# Autodesk Inventor assembly: 00_033_BATTERY_LIB_R1
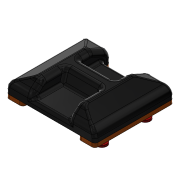
[picture p0: Inventor's stored thumbnail of the model, 180x180]
Saved by Autodesk Inventor 2021.2 (Build 252289000, 289)
## iProperties
Created: 2018-09-07
Part Number: 00_033_BATTERY_LIB_R1
Material: 一般
Document SubType Name: Assembly
Designer: y6tada
Author: y6tada
## Documents named in this file (4)
- C:\Workspace\HaptHexa\Hardware\Inventor\00_033_BATTERY_LIB_R1.iam
- C:\Workspace\HaptHexa\Hardware\Inventor\15_037_BATTERY_LIB_OUTER_R1.ipt
- C:\Workspace\HaptHexa\Hardware\Inventor\10_036_BATTERY_COVER_BASE_R1.ipt
- C:\Workspace\HaptHexa\Hardware\Inventor\16_038_BATTERY_LIB_HOOK_R1.ipt
## Components (3 placed, 3 different names)
1. battery_cover_base:1 — メイト:1, フラッシュ:1, メイト:2, メイト:3, フラッシュ:2, メイト:4, フラッシュ:3, フラッシュ:5
2. battery_lid_print:1 — メイト:3, フラッシュ:2, メイト:4
3. battery_lib_hook:1 — フラッシュ:3, メイト:5, フラッシュ:4, フラッシュ:5
## Relationships (10: Mate 5, Flush 5)
- メイト:1 [Mate]: battery_cover_base:1
- フラッシュ:1 [Flush]: battery_cover_base:1
- メイト:2 [Mate]: battery_cover_base:1
- メイト:3 [Mate]: battery_cover_base:1 ↔ battery_lid_print:1
- フラッシュ:2 [Flush]: battery_cover_base:1 ↔ battery_lid_print:1
- メイト:4 [Mate]: battery_cover_base:1 ↔ battery_lid_print:1
- フラッシュ:3 [Flush]: battery_cover_base:1 ↔ battery_lib_hook:1
- メイト:5 [Mate]: battery_lib_hook:1
- フラッシュ:4 [Flush]: battery_lib_hook:1
- フラッシュ:5 [Flush]: battery_cover_base:1 ↔ battery_lib_hook:1
